# Autodesk Inventor assembly: Gantry
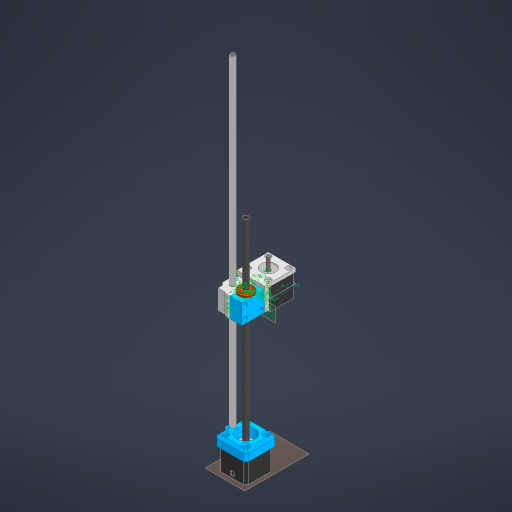
[picture p0: Inventor's stored thumbnail of the model, 512x512]
Saved by Autodesk Inventor 2024.2 (Build 282272000, 272)
## iProperties
Created: 2024-10-02
Part Number: Gantry
Document SubType Name: Assembly
Designer: jerem
Author: jerem
## Documents named in this file (9)
- C:\Users\jerem\Documents\GitHub\Perovskite-Automated-Synthesis-System\CAD\Gantry\Gantry.iam
- C:\Users\jerem\Documents\GitHub\Perovskite-Automated-Synthesis-System\CAD\Gantry\Reference\NEMA17 Stepper Motor.ipt
- C:\Users\jerem\Documents\GitHub\Perovskite-Automated-Synthesis-System\CAD\Gantry\Stepper Holder.ipt
- C:\Users\jerem\Documents\GitHub\Perovskite-Automated-Synthesis-System\CAD\Gantry\Reference\Linear Rod 8mm x 500mm.ipt
- C:\Users\jerem\Documents\GitHub\Perovskite-Automated-Synthesis-System\CAD\Gantry\Reference\Linear Bearing 8mm Square.ipt
- C:\Users\jerem\Documents\GitHub\Perovskite-Automated-Synthesis-System\CAD\Gantry\Reference\Leadscrew.ipt
- C:\Users\jerem\Documents\GitHub\Perovskite-Automated-Synthesis-System\CAD\Gantry\ZX Axis Carriage.ipt
- C:\Users\jerem\Documents\GitHub\Perovskite-Automated-Synthesis-System\CAD\Gantry\Reference\Threaded Rod 300mm.ipt
- C:\Users\jerem\Documents\GitHub\Perovskite-Automated-Synthesis-System\CAD\Gantry\CoreXY Stepper Holder.ipt
## Components (9 placed, 8 different names)
1. NEMA17 Stepper Motor:1 — Mate:1, Mate:2, Mate:3, Mate:7, Mate:71, Mate:72
2. Stepper Holder:1 — Mate:1, Mate:2, Mate:3, Mate:4, Mate:5
3. Linear Rod 8mm x 500mm:1 — Mate:4, Mate:5, Mate:6
4. Linear Bearing 8mm Square:1 — Mate:6, Mate:73
5. Leadscrew:1 — Mate:7, Mate:10, Mate:11, Mate:12
6. ZX Axis Carriage:1 — Mate:10, Mate:11, Mate:12, Mate:73, Mate:74, Mate:75, Mate:80
7. Threaded Rod 300mm:1 — Mate:71, Mate:72
8. CoreXY Stepper Holder:1 — Mate:74, Mate:75, Mate:77, Mate:78, Mate:79, Mate:80
9. NEMA17 Stepper Motor:2 — Mate:77, Mate:78, Mate:79
## Relationships (19: Mate 19)
- Mate:1: NEMA17 Stepper Motor:1 ↔ Stepper Holder:1
- Mate:2: NEMA17 Stepper Motor:1 ↔ Stepper Holder:1
- Mate:3: NEMA17 Stepper Motor:1 ↔ Stepper Holder:1
- Mate:4: Stepper Holder:1 ↔ Linear Rod 8mm x 500mm:1
- Mate:5: Stepper Holder:1 ↔ Linear Rod 8mm x 500mm:1
- Mate:6: Linear Rod 8mm x 500mm:1 ↔ Linear Bearing 8mm Square:1
- Mate:7: NEMA17 Stepper Motor:1 ↔ Leadscrew:1
- Mate:10: Leadscrew:1 ↔ ZX Axis Carriage:1
- Mate:11: Leadscrew:1 ↔ ZX Axis Carriage:1
- Mate:12: Leadscrew:1 ↔ ZX Axis Carriage:1
- Mate:71: NEMA17 Stepper Motor:1 ↔ Threaded Rod 300mm:1
- Mate:72: NEMA17 Stepper Motor:1 ↔ Threaded Rod 300mm:1
- Mate:73: Linear Bearing 8mm Square:1 ↔ ZX Axis Carriage:1
- Mate:74: ZX Axis Carriage:1 ↔ CoreXY Stepper Holder:1
- Mate:75: ZX Axis Carriage:1 ↔ CoreXY Stepper Holder:1
- Mate:77: CoreXY Stepper Holder:1 ↔ NEMA17 Stepper Motor:2
- Mate:78: CoreXY Stepper Holder:1 ↔ NEMA17 Stepper Motor:2
- Mate:79: CoreXY Stepper Holder:1 ↔ NEMA17 Stepper Motor:2
- Mate:80: ZX Axis Carriage:1 ↔ CoreXY Stepper Holder:1
